# Autodesk Inventor assembly: Radius Gauge Case
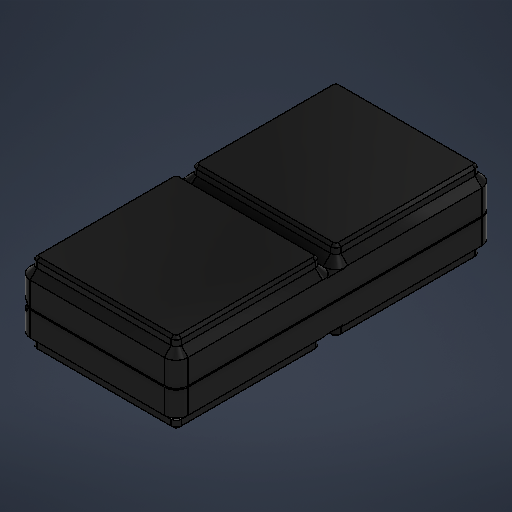
[picture p0: Inventor's stored thumbnail of the model, 512x512]
Saved by Autodesk Inventor 2026.1 (Build 301233020, 233B)
## iProperties
Created: 2025-10-25
Part Number: Radius Gauge Case
Document SubType Name: Assembly
Designer: JoshuaEah
Author: JoshuaEah
## Documents named in this file (3)
- C:\Users\JoshuaEah\Documents\GitHub\Designed-Trinkets\Radius Gauge\Radius Gauge Case.iam
- C:\Users\JoshuaEah\Documents\GitHub\Designed-Trinkets\Radius Gauge\Radius Gauge Case (Lower).ipt
- C:\Users\JoshuaEah\Documents\GitHub\Designed-Trinkets\Radius Gauge\Radius Gauge Case (Upper).ipt
## Components (2 placed, 2 different names)
1. Radius Gauge Case (Lower):1 — Mate:1, Angle:1, Mate:2, Flush:1
2. Radius Gauge Case (Upper):1 — Angle:1, Mate:2, Flush:1
## Relationships (4: Mate 2, Angle 1, Flush 1)
- Mate:1: Radius Gauge Case (Lower):1
- Angle:1 (180 deg): Radius Gauge Case (Lower):1 ↔ Radius Gauge Case (Upper):1
- Mate:2: Radius Gauge Case (Lower):1 ↔ Radius Gauge Case (Upper):1
- Flush:1: Radius Gauge Case (Lower):1 ↔ Radius Gauge Case (Upper):1
